# Autodesk Inventor assembly: dcbuddy_v2
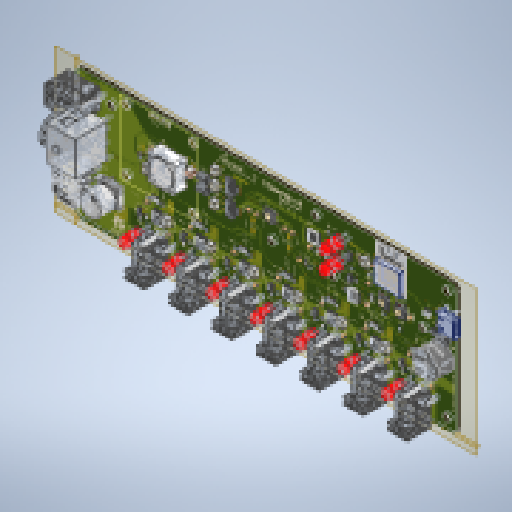
[picture p0: Inventor's stored thumbnail of the model, 512x512]
Saved by Autodesk Inventor 2024.3 (Build 283343000, 343)
## iProperties
Created: 2024-05-05
Part Number: dcbuddy_v2
Document SubType Name: Assembly
Designer: atrus
Author: atrus
## Documents named in this file (36)
- C:\Users\atrus\Dropbox\elec\Mechanical\DCBuddyV2\PCB\dcbuddy_v2.iam
- C:\Users\atrus\Dropbox\elec\Mechanical\DCBuddyV2\PCB\dcbuddy_v2_BOARD.ipt
- C:\Users\atrus\Dropbox\elec\Mechanical\DCBuddyV2\PCB\ConvertedComponents\RESC1608-IPC-ML_CMP-009-00191-4.ipt
- C:\Users\atrus\Dropbox\elec\Mechanical\DCBuddyV2\PCB\ConvertedComponents\OLED_1_3_CARRIERBOARD-Footprint-1_CMP-00028-00008-2.ipt
- C:\Users\atrus\Dropbox\elec\Mechanical\DCBuddyV2\PCB\ConvertedComponents\FP-D0008A-IPC_B_CMP-015-00015-1.ipt
- C:\Users\atrus\Dropbox\elec\Mechanical\DCBuddyV2\PCB\ConvertedComponents\RESC1608-IPC-ML_CMP-009-00069-2.ipt
- C:\Users\atrus\Dropbox\elec\Mechanical\DCBuddyV2\PCB\ConvertedComponents\FP-CL10-IPC_B_CMP-001-00084-7.ipt
- C:\Users\atrus\Dropbox\elec\Mechanical\DCBuddyV2\PCB\ConvertedComponents\DCY0004A_M_CMP-019-00080-1.ipt
- C:\Users\atrus\Dropbox\elec\Mechanical\DCBuddyV2\PCB\ConvertedComponents\LED5MM_CMP-130-0003-6.ipt
- C:\Users\atrus\Dropbox\elec\Mechanical\DCBuddyV2\PCB\ConvertedComponents\DCY0004A_M_CMP-019-00078-1.ipt
- C:\Users\atrus\Dropbox\elec\Mechanical\DCBuddyV2\PCB\ConvertedComponents\SOT95P280X145-6N_CMP-019-00077-1.ipt
- C:\Users\atrus\Dropbox\elec\Mechanical\DCBuddyV2\PCB\ConvertedComponents\PW0016A_L_CMP-015-00016-1.ipt
- C:\Users\atrus\Dropbox\elec\Mechanical\DCBuddyV2\PCB\ConvertedComponents\XCVR_ESP32-C3-MINI-1-N4_CMP-206-000000-1.ipt
- C:\Users\atrus\Dropbox\elec\Mechanical\DCBuddyV2\PCB\ConvertedComponents\FP-PWP0014C-IPC_C_CMP-024-00009-1.ipt
- C:\Users\atrus\Dropbox\elec\Mechanical\DCBuddyV2\PCB\ConvertedComponents\FP-PTS526SK15SMTR2LFS-MFG_CMP-011-00015-1.ipt
- C:\Users\atrus\Dropbox\elec\Mechanical\DCBuddyV2\PCB\ConvertedComponents\RESC1608X55X30NL20T20_CMP-009-00235-1.ipt
- C:\Users\atrus\Dropbox\elec\Mechanical\DCBuddyV2\PCB\ConvertedComponents\RESC1608-IPC-LL_CMP-009-00203-1.ipt
- C:\Users\atrus\Dropbox\elec\Mechanical\DCBuddyV2\PCB\ConvertedComponents\FP-AC0402-IPC_A_CMP-009-00234-1.ipt
- C:\Users\atrus\Dropbox\elec\Mechanical\DCBuddyV2\PCB\ConvertedComponents\RESC1608-IPC-ML_CMP-009-00183-3.ipt
- C:\Users\atrus\Dropbox\elec\Mechanical\DCBuddyV2\PCB\ConvertedComponents\RESC1608-IPC-ML_CMP-009-00205-1.ipt
- C:\Users\atrus\Dropbox\elec\Mechanical\DCBuddyV2\PCB\ConvertedComponents\RESC2013X60X35LL10T20_CMP-009-00233-1.ipt
- C:\Users\atrus\Dropbox\elec\Mechanical\DCBuddyV2\PCB\ConvertedComponents\RESC1608-IPC-LL_CMP-009-00222-1.ipt
- C:\Users\atrus\Dropbox\elec\Mechanical\DCBuddyV2\PCB\ConvertedComponents\SOT23-3_CMP-094-0000-1.ipt
- C:\Users\atrus\Dropbox\elec\Mechanical\DCBuddyV2\PCB\ConvertedComponents\SRR1260-680M-Footprint-1_CMP-006-00034-1.ipt
- C:\Users\atrus\Dropbox\elec\Mechanical\DCBuddyV2\PCB\ConvertedComponents\CUI-PJ-002A_V_CMP-167-0003-2.ipt
- C:\Users\atrus\Dropbox\elec\Mechanical\DCBuddyV2\PCB\ConvertedComponents\PD40S_CMP-167-0005-1.ipt
- C:\Users\atrus\Dropbox\elec\Mechanical\DCBuddyV2\PCB\ConvertedComponents\AMPHENOL_10155435-00011LF_CMP-243-000000-3.ipt
- C:\Users\atrus\Dropbox\elec\Mechanical\DCBuddyV2\PCB\ConvertedComponents\SMA_CMP-080-0002-2.ipt
- C:\Users\atrus\Dropbox\elec\Mechanical\DCBuddyV2\PCB\ConvertedComponents\FP-SOT23-6L-MFG_CMP-004-00040-1.ipt
- C:\Users\atrus\Dropbox\elec\Mechanical\DCBuddyV2\PCB\ConvertedComponents\FP-FKG-MFG_CMP-001-00124-1.ipt
- C:\Users\atrus\Dropbox\elec\Mechanical\DCBuddyV2\PCB\ConvertedComponents\CAPC3225X20N_CMP-001-00083-3.ipt
- C:\Users\atrus\Dropbox\elec\Mechanical\DCBuddyV2\PCB\ConvertedComponents\FP-1210-L_3_2_0_3-W_2_5_0-MFG_CMP-001-00125-1.ipt
- C:\Users\atrus\Dropbox\elec\Mechanical\DCBuddyV2\PCB\ConvertedComponents\FP-CL10-IPC_C_CMP-001-00101-4.ipt
- C:\Users\atrus\Dropbox\elec\Mechanical\DCBuddyV2\PCB\ConvertedComponents\FP-CL10-IPC_B_CMP-001-00085-7.ipt
- C:\Users\atrus\Dropbox\elec\Mechanical\DCBuddyV2\PCB\ConvertedComponents\WST-1212UX-Footprint-1_CMP-00027-00003-3.ipt
- C:\Users\atrus\Dropbox\elec\Mechanical\DCBuddyV2\PCB\ConvertedComponents\FP-43045-0802-MFG_CMP-002-00102-1.ipt
## Components (161 placed, 35 different names)
1. dcbuddy_v2_BOARD:1 — Flush:1
2. RESC1608-IPC-ML_CMP-009-00191-4:1
3. RESC1608-IPC-ML_CMP-009-00191-4:2
4. RESC1608-IPC-ML_CMP-009-00191-4:3
5. RESC1608-IPC-ML_CMP-009-00191-4:4
6. RESC1608-IPC-ML_CMP-009-00191-4:5
7. RESC1608-IPC-ML_CMP-009-00191-4:6
8. RESC1608-IPC-ML_CMP-009-00191-4:7
9. OLED_1_3_CARRIERBOARD-Footprint-1_CMP-00028-00008-2:1
10. FP-D0008A-IPC_B_CMP-015-00015-1:1
11. RESC1608-IPC-ML_CMP-009-00069-2:1
12. FP-CL10-IPC_B_CMP-001-00084-7:1
13. FP-CL10-IPC_B_CMP-001-00084-7:2
14. FP-CL10-IPC_B_CMP-001-00084-7:3
15. FP-CL10-IPC_B_CMP-001-00084-7:6
16. FP-CL10-IPC_B_CMP-001-00084-7:7
17. FP-CL10-IPC_B_CMP-001-00084-7:8
18. FP-CL10-IPC_B_CMP-001-00084-7:23
19. DCY0004A_M_CMP-019-00080-1:1
20. LED5MM_CMP-130-0003-6:1
21. LED5MM_CMP-130-0003-6:2
22. DCY0004A_M_CMP-019-00078-1:1
23. SOT95P280X145-6N_CMP-019-00077-1:1
24. PW0016A_L_CMP-015-00016-1:1
25. XCVR_ESP32-C3-MINI-1-N4_CMP-206-000000-1:1
26. FP-PTS526SK15SMTR2LFS-MFG_CMP-011-00015-1:1
27. FP-PTS526SK15SMTR2LFS-MFG_CMP-011-00015-1:2
28. RESC1608X55X30NL20T20_CMP-009-00235-1:1
29. RESC1608X55X30NL20T20_CMP-009-00235-1:2
30. RESC1608-IPC-LL_CMP-009-00203-1:1
31. FP-AC0402-IPC_A_CMP-009-00234-1:1
32. FP-AC0402-IPC_A_CMP-009-00234-1:2
33. RESC1608-IPC-ML_CMP-009-00183-3:1
34. RESC1608-IPC-ML_CMP-009-00183-3:2
35. RESC1608-IPC-LL_CMP-009-00222-1:1
36. SOT23-3_CMP-094-0000-1:1
37. SOT23-3_CMP-094-0000-1:2
38. SRR1260-680M-Footprint-1_CMP-006-00034-1:1
39. CUI-PJ-002A_V_CMP-167-0003-2:1
40. PD40S_CMP-167-0005-1:1
41. AMPHENOL_10155435-00011LF_CMP-243-000000-3:1
42. SMA_CMP-080-0002-2:1
43. SMA_CMP-080-0002-2:2
44. FP-SOT23-6L-MFG_CMP-004-00040-1:1
45. FP-FKG-MFG_CMP-001-00124-1:1
46. CAPC3225X20N_CMP-001-00083-3:1
47. CAPC3225X20N_CMP-001-00083-3:2
48. CAPC3225X20N_CMP-001-00083-3:3
49. CAPC3225X20N_CMP-001-00083-3:4
50. CAPC3225X20N_CMP-001-00083-3:5
51. FP-1210-L_3_2_0_3-W_2_5_0-MFG_CMP-001-00125-1:1
52. FP-CL10-IPC_B_CMP-001-00085-7:1
53. FP-CL10-IPC_B_CMP-001-00085-7:2
54. WST-1212UX-Footprint-1_CMP-00027-00003-3:1
55. SOT23-3_CMP-094-0000-1:3
56. SOT23-3_CMP-094-0000-1:4
57. SOT23-3_CMP-094-0000-1:5
58. SOT23-3_CMP-094-0000-1:6
59. SOT23-3_CMP-094-0000-1:7
60. SOT23-3_CMP-094-0000-1:8
61. SOT23-3_CMP-094-0000-1:9
62. SOT23-3_CMP-094-0000-1:10
63. SMA_CMP-080-0002-2:3
64. RESC1608-IPC-ML_CMP-009-00191-4:8
65. RESC1608-IPC-ML_CMP-009-00191-4:9
66. RESC1608-IPC-ML_CMP-009-00191-4:10
67. RESC1608-IPC-ML_CMP-009-00191-4:11
68. RESC1608-IPC-ML_CMP-009-00191-4:12
69. RESC1608-IPC-ML_CMP-009-00191-4:13
70. RESC1608-IPC-ML_CMP-009-00191-4:14
71. RESC1608-IPC-ML_CMP-009-00191-4:15
72. FP-PTS526SK15SMTR2LFS-MFG_CMP-011-00015-1:3
73. FP-CL10-IPC_B_CMP-001-00084-7:24
74. FP-CL10-IPC_B_CMP-001-00084-7:25
75. FP-CL10-IPC_B_CMP-001-00084-7:26
76. FP-CL10-IPC_B_CMP-001-00084-7:27
77. FP-CL10-IPC_B_CMP-001-00084-7:28
78. FP-CL10-IPC_B_CMP-001-00084-7:29
79. FP-CL10-IPC_B_CMP-001-00084-7:30
80. FP-CL10-IPC_B_CMP-001-00084-7:31
81. FP-CL10-IPC_B_CMP-001-00084-7:32
82. FP-CL10-IPC_B_CMP-001-00084-7:33
83. FP-CL10-IPC_B_CMP-001-00084-7:34
84. FP-CL10-IPC_B_CMP-001-00084-7:35
85. FP-CL10-IPC_B_CMP-001-00084-7:36
86. FP-CL10-IPC_B_CMP-001-00084-7:37
87. FP-CL10-IPC_B_CMP-001-00084-7:38
88. FP-CL10-IPC_B_CMP-001-00084-7:39
89. FP-43045-0802-MFG_CMP-002-00102-1:1
90. LED5MM_CMP-130-0003-6:3
91. LED5MM_CMP-130-0003-6:4
92. LED5MM_CMP-130-0003-6:5
93. LED5MM_CMP-130-0003-6:6
94. LED5MM_CMP-130-0003-6:7
95. LED5MM_CMP-130-0003-6:8
96. LED5MM_CMP-130-0003-6:9
97. FP-PWP0014C-IPC_C_CMP-024-00009-1:1
98. FP-PWP0014C-IPC_C_CMP-024-00009-1:2
99. FP-PWP0014C-IPC_C_CMP-024-00009-1:3
100. FP-PWP0014C-IPC_C_CMP-024-00009-1:4
101. FP-PWP0014C-IPC_C_CMP-024-00009-1:5
102. FP-PWP0014C-IPC_C_CMP-024-00009-1:6
103. FP-PWP0014C-IPC_C_CMP-024-00009-1:7
104. RESC1608-IPC-ML_CMP-009-00183-3:3
105. RESC1608-IPC-ML_CMP-009-00183-3:4
106. RESC1608-IPC-ML_CMP-009-00183-3:5
107. RESC1608-IPC-ML_CMP-009-00183-3:6
108. RESC1608-IPC-ML_CMP-009-00183-3:7
109. RESC1608-IPC-ML_CMP-009-00183-3:8
110. RESC1608-IPC-ML_CMP-009-00183-3:9
111. RESC1608-IPC-ML_CMP-009-00205-1:1
112. RESC1608-IPC-ML_CMP-009-00205-1:2
113. RESC1608-IPC-ML_CMP-009-00205-1:3
114. RESC1608-IPC-ML_CMP-009-00205-1:4
115. RESC1608-IPC-ML_CMP-009-00205-1:5
116. RESC1608-IPC-ML_CMP-009-00205-1:6
117. RESC1608-IPC-ML_CMP-009-00205-1:7
118. RESC1608-IPC-ML_CMP-009-00205-1:8
119. RESC1608-IPC-ML_CMP-009-00205-1:9
120. RESC1608-IPC-ML_CMP-009-00205-1:10
121. RESC1608-IPC-ML_CMP-009-00205-1:11
122. RESC1608-IPC-ML_CMP-009-00205-1:12
123. RESC1608-IPC-ML_CMP-009-00205-1:13
124. RESC1608-IPC-ML_CMP-009-00205-1:14
125. RESC1608-IPC-ML_CMP-009-00205-1:15
126. RESC1608-IPC-ML_CMP-009-00205-1:16
127. RESC1608-IPC-ML_CMP-009-00205-1:17
128. RESC1608-IPC-ML_CMP-009-00205-1:18
129. RESC1608-IPC-ML_CMP-009-00205-1:19
130. RESC1608-IPC-ML_CMP-009-00205-1:20
131. RESC1608-IPC-ML_CMP-009-00205-1:21
132. RESC2013X60X35LL10T20_CMP-009-00233-1:1
133. RESC2013X60X35LL10T20_CMP-009-00233-1:2
134. RESC2013X60X35LL10T20_CMP-009-00233-1:3
135. RESC2013X60X35LL10T20_CMP-009-00233-1:4
136. RESC2013X60X35LL10T20_CMP-009-00233-1:5
137. RESC2013X60X35LL10T20_CMP-009-00233-1:6
138. RESC2013X60X35LL10T20_CMP-009-00233-1:7
139. RESC2013X60X35LL10T20_CMP-009-00233-1:8
140. RESC2013X60X35LL10T20_CMP-009-00233-1:9
141. RESC2013X60X35LL10T20_CMP-009-00233-1:10
142. RESC2013X60X35LL10T20_CMP-009-00233-1:11
143. RESC2013X60X35LL10T20_CMP-009-00233-1:12
144. RESC2013X60X35LL10T20_CMP-009-00233-1:13
145. RESC2013X60X35LL10T20_CMP-009-00233-1:14
146. CUI-PJ-002A_V_CMP-167-0003-2:2
147. CUI-PJ-002A_V_CMP-167-0003-2:3
148. CUI-PJ-002A_V_CMP-167-0003-2:4
149. CUI-PJ-002A_V_CMP-167-0003-2:5
150. CUI-PJ-002A_V_CMP-167-0003-2:6
151. CUI-PJ-002A_V_CMP-167-0003-2:7
152. CUI-PJ-002A_V_CMP-167-0003-2:8
153. CAPC3225X20N_CMP-001-00083-3:6
154. CAPC3225X20N_CMP-001-00083-3:7
155. CAPC3225X20N_CMP-001-00083-3:8
156. CAPC3225X20N_CMP-001-00083-3:9
157. CAPC3225X20N_CMP-001-00083-3:10
158. CAPC3225X20N_CMP-001-00083-3:11
159. CAPC3225X20N_CMP-001-00083-3:12
160. FP-CL10-IPC_C_CMP-001-00101-4:1
161. FP-CL10-IPC_C_CMP-001-00101-4:2
## Relationships (1: Flush 1)
- Flush:1 (0.1 mm): dcbuddy_v2_BOARD:1
